# Autodesk Inventor assembly: Сборка1
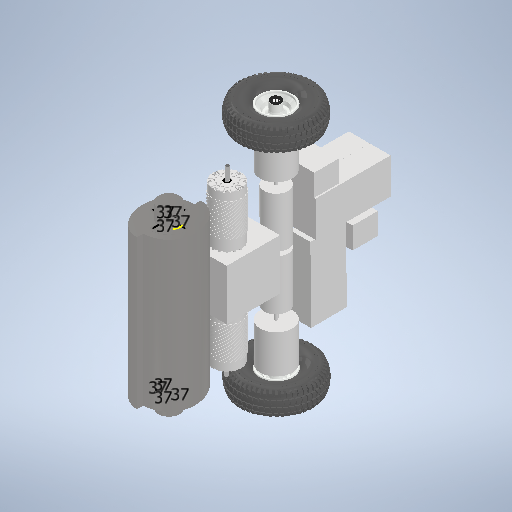
[picture p0: Inventor's stored thumbnail of the model, 512x512]
Saved by Autodesk Inventor 2025.1 (Build 291241000, 241)
## iProperties
Created: 2025-04-09
Part Number: Сборка1
Document SubType Name: Assembly
Designer: tishk
Author: tishk
## Documents named in this file (10)
- C:\Users\tishk\Desktop\Projects\Битва роботов\BOBR\BOBR\Сборка1.iam
- C:\Users\tishk\Desktop\Projects\Битва роботов\BOBR\BOBR\Спиннер.ipt
- C:\Users\tishk\Desktop\Projects\Битва роботов\BOBR\BOBR\КреплениеБарабана.ipt
- C:\Users\tishk\Desktop\Projects\Битва роботов\BOBR\BOBR\Hobbywing EZrun max4.ipt
- C:\Users\tishk\Desktop\Projects\Битва роботов\BOBR\BOBR\Hobbywing EZrun max5.ipt
- C:\Users\tishk\Desktop\Projects\Битва роботов\BOBR\BOBR\Контроллер EZrun max4.ipt
- C:\Users\tishk\Desktop\Projects\Битва роботов\BOBR\BOBR\Контроллер EZrun max5.ipt
- C:\Users\tishk\Desktop\Projects\Битва роботов\BOBR\BOBR\Lipo Battery 9500mAh 29.6V.ipt
- C:\Users\tishk\Desktop\Projects\Битва роботов\BOBR\BOBR\Редуктор (прикидка).ipt
- C:\Users\tishk\Desktop\Projects\Битва роботов\BOBR\BOBR\колесо.ipt
## Components (18 placed, 9 different names)
1. Спиннер:1 — Совмещение:1, Совмещение:2, Совмещение:3, Совмещение:4, Совмещение:5, Совмещение:6
2. КреплениеБарабана:1 — Совмещение:4, Совмещение:5, Совмещение:6
3. КреплениеБарабана:2 — Совмещение:1, Совмещение:2, Совмещение:3
4. Hobbywing EZrun max4:1 — Совмещение:25
5. Hobbywing EZrun max4:2 — Совмещение:25
6. Hobbywing EZrun max5:4 — Совмещение:8, Совмещение:9
7. Контроллер EZrun max4:1 — Заподлицо:11, Заподлицо:12
8. Контроллер EZrun max4:2 — Заподлицо:11, Заподлицо:12
9. Контроллер EZrun max5:4 — Заподлицо:10, Совмещение:29
10. Lipo Battery 9500mAh 29.6V:1
11. Lipo Battery 9500mAh 29.6V:2 — Совмещение:7, Заподлицо:1, Заподлицо:2
12. Lipo Battery 9500mAh 29.6V:3 — Совмещение:7, Заподлицо:1, Заподлицо:2, Заподлицо:10, Совмещение:29
13. Редуктор (прикидка):2 — Совмещение:8, Совмещение:9, Совмещение:22, Совмещение:23
14. колесо:2 — Совмещение:22, Совмещение:23
15. Hobbywing EZrun max5:7
16. Редуктор (прикидка):5
17. колесо:5
18. Контроллер EZrun max5:5
## Relationships (22: Mate 17, Flush 5)
- Совмещение:1 [Mate]: Спиннер:1 ↔ КреплениеБарабана:2
- Совмещение:2 [Mate]: Спиннер:1 ↔ КреплениеБарабана:2
- Совмещение:3 [Mate]: Спиннер:1 ↔ КреплениеБарабана:2
- Совмещение:4 [Mate]: Спиннер:1 ↔ КреплениеБарабана:1
- Совмещение:5 [Mate]: Спиннер:1 ↔ КреплениеБарабана:1
- Совмещение:6 [Mate]: Спиннер:1 ↔ КреплениеБарабана:1
- Совмещение:7 [Mate]: Lipo Battery 9500mAh 29.6V:2 ↔ Lipo Battery 9500mAh 29.6V:3
- Заподлицо:1 [Flush]: Lipo Battery 9500mAh 29.6V:2 ↔ Lipo Battery 9500mAh 29.6V:3
- Заподлицо:2 [Flush]: Lipo Battery 9500mAh 29.6V:2 ↔ Lipo Battery 9500mAh 29.6V:3
- Совмещение:8 [Mate]: Hobbywing EZrun max5:4 ↔ Редуктор (прикидка):2
- Совмещение:9 [Mate]: Hobbywing EZrun max5:4 ↔ Редуктор (прикидка):2
- Совмещение:22 [Mate]: Редуктор (прикидка):2 ↔ колесо:2
- Совмещение:23 [Mate]: Редуктор (прикидка):2 ↔ колесо:2
- Совмещение:25 [Mate]: Hobbywing EZrun max4:1 ↔ Hobbywing EZrun max4:2
- Заподлицо:10 [Flush]: Контроллер EZrun max5:4 ↔ Lipo Battery 9500mAh 29.6V:3
- Совмещение:29 [Mate]: Контроллер EZrun max5:4 ↔ Lipo Battery 9500mAh 29.6V:3
- Заподлицо:11 [Flush]: Контроллер EZrun max4:1 ↔ Контроллер EZrun max4:2
- Заподлицо:12 [Flush]: Контроллер EZrun max4:1 ↔ Контроллер EZrun max4:2
- [Mate]: Hobbywing EZrun max5:7 ↔ Редуктор (прикидка):5
- [Mate]: Hobbywing EZrun max5:7 ↔ Редуктор (прикидка):5
- [Mate]: Редуктор (прикидка):5 ↔ колесо:5
- [Mate]: Редуктор (прикидка):5 ↔ колесо:5
## Named parameters: d50_d46_d9 = 0 mm, d51_d47_d10 = 0 mm, d52_d48_d23 = 0 mm, d53_d49_d24 = 0 mm
